# Autodesk Inventor assembly: s-assy-spacer1
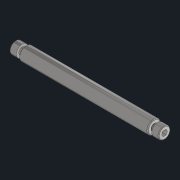
[picture p0: Inventor's stored thumbnail of the model, 180x180]
Saved by Autodesk Inventor 2021 (Build 250183000, 183)
## iProperties
Created: 2021-08-04
Part Number: s-assy-spacer1
Document SubType Name: Assembly
Designer: yuta0
Author: yuta0
## Documents named in this file (3)
- C:\Users\yuta0\Desktop\catchrobo_robot\s-assy-spacer1.iam
- C:\Users\yuta0\Desktop\lab\nicebot\CB4-10.ipt
- C:\Users\yuta0\Desktop\catchrobo_robot\SFHRW8-76-M4-N4.ipt
## Components (3 placed, 2 different names)
1. SFHRW8-76-M4-N4:1
2. CB4-10:1
3. CB4-10:2
## Relationships (4: Mate 4)
- [Mate]: SFHRW8-76-M4-N4:1 ↔ CB4-10:2
- [Mate]: SFHRW8-76-M4-N4:1 ↔ CB4-10:1
- [Mate] (2 mm): SFHRW8-76-M4-N4:1 ↔ CB4-10:1
- [Mate] (2 mm): SFHRW8-76-M4-N4:1 ↔ CB4-10:2
